# Autodesk Inventor assembly: Dynamic_Hinge
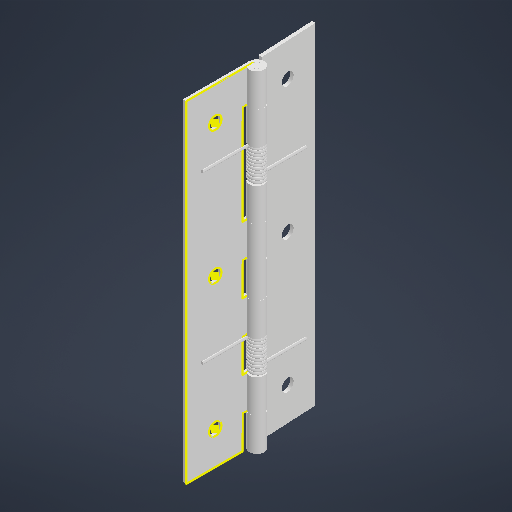
[picture p0: Inventor's stored thumbnail of the model, 512x512]
Saved by Autodesk Inventor 2026.2 (Build 302298010, 298A)
## iProperties
Created: 2026-06-02
Part Number: Dynamic_Hinge
Document SubType Name: Assembly
Designer: Srishanth Dhondy
Author: Srishanth Dhondy
## Documents named in this file (6)
- D:\Cloud_Downloads\Srishanth\My Folder\Projects\AMR\CAD Design\hardware_cad\15205A113_Spring Hinge\15205A113_Spring Hinge\Dynamic_Hinge.iam
- D:\Cloud_Downloads\Srishanth\My Folder\Projects\AMR\CAD Design\hardware_cad\15205A113_Spring Hinge\15205A113_Spring Hinge\Solid1.ipt
- D:\Cloud_Downloads\Srishanth\My Folder\Projects\AMR\CAD Design\hardware_cad\15205A113_Spring Hinge\15205A113_Spring Hinge\Solid2.ipt
- D:\Cloud_Downloads\Srishanth\My Folder\Projects\AMR\CAD Design\hardware_cad\15205A113_Spring Hinge\15205A113_Spring Hinge\Solid3.ipt
- D:\Cloud_Downloads\Srishanth\My Folder\Projects\AMR\CAD Design\hardware_cad\15205A113_Spring Hinge\15205A113_Spring Hinge\Solid4.ipt
- D:\Cloud_Downloads\Srishanth\My Folder\Projects\AMR\CAD Design\hardware_cad\15205A113_Spring Hinge\15205A113_Spring Hinge\Solid5.ipt
## Components (5 placed, 5 different names)
1. Solid1:1 — Cylindrical:1
2. Solid2:1
3. Solid3:1 — Mate:1
4. Solid4:1 — Cylindrical:1, Mate:1
5. Solid5:1
## Relationships (2: CylindricalJoint 1, Mate 1)
- Cylindrical:1: Solid1:1 ↔ Solid4:1
- Mate:1: Solid3:1 ↔ Solid4:1
